# Autodesk Inventor assembly: servo and arm
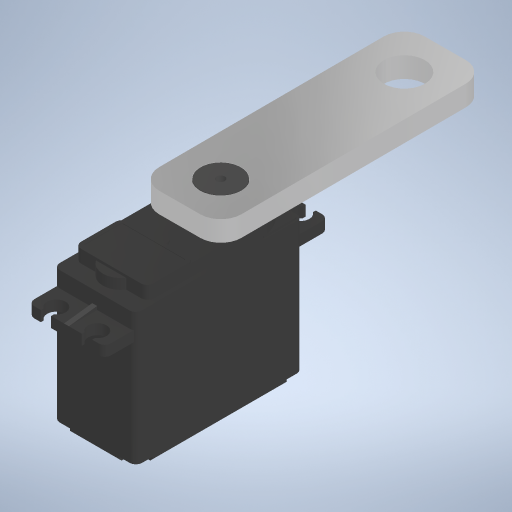
[picture p0: Inventor's stored thumbnail of the model, 512x512]
Saved by Autodesk Inventor 2023 (Build 270158000, 158)
## iProperties
Created: 2022-06-23
Part Number: servo and arm
Document SubType Name: Assembly
Designer: earls
Author: earls
## Documents named in this file (3)
- F:\Documents\Mechatronic Engineering 5.1\Project\CAD\servo and arm.iam
- F:\Documents\Mechatronic Engineering 5.1\Project\CAD\ServoMotor\Servo.ipt
- F:\Documents\Mechatronic Engineering 5.1\Project\CAD\Servo arm.ipt
## Components (2 placed, 2 different names)
1. Servo:1 — Rotational:1
2. Servo arm:1 — Rotational:1
## Relationships (1: RevoluteJoint 1)
- Rotational:1 [RevoluteJoint]: Servo:1 ↔ Servo arm:1
